# Autodesk Inventor assembly: Assembly1
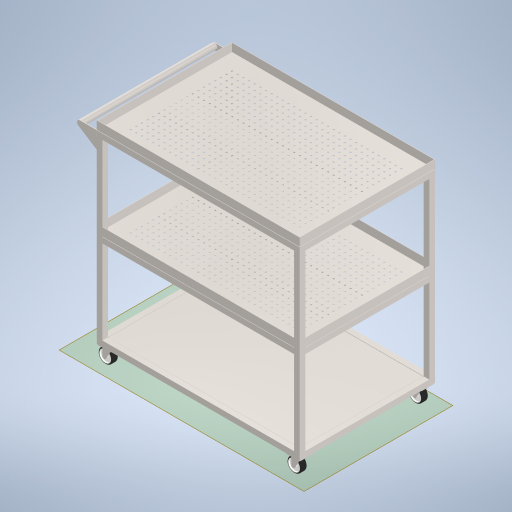
[picture p0: Inventor's stored thumbnail of the model, 512x512]
Saved by Autodesk Inventor 2023 (Build 270158000, 158)
## iProperties
Created: 2023-03-07
Part Number: Assembly1
Document SubType Name: Assembly
Designer: klebe
Author: klebe
## Documents named in this file (2)
- C:\Users\klebe\OneDrive\Documents\GitHub\Sala-braquiterapia\Sala de Braquiterapia\Inventor\mesa\Assembly1.iam
- C:\Users\klebe\OneDrive\Documents\GitHub\Sala-braquiterapia\Sala de Braquiterapia\Inventor\mesa\ss-service-table-1.snapshot.2\service table.ipt
## Components (1 placed, 1 different names)
1. service table:1 — Flush:1, Mate:1, Mate:2
## Relationships (3: Mate 2, Flush 1)
- Flush:1: service table:1
- Mate:1: service table:1
- Mate:2: service table:1
